# Autodesk Inventor assembly: AM14U3 Long Frame Half
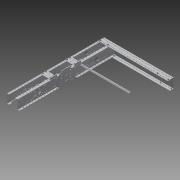
[picture p0: Inventor's stored thumbnail of the model, 180x180]
Saved by Autodesk Inventor 2018 (Build 220112000, 112)
## iProperties
Created: 2015-12-05
Part Number: AM14U3 Long Frame Half
Document SubType Name: Assembly
Designer: PhillipD
Author: PhillipD
Revision Number: ANY
## Documents named in this file (9)
- D:\FIRST 2018\FIRST 2018 Inventor\FIRST 2017 Drive Base\Parts\AM14U3 Long Frame Half.iam
- D:\FIRST 2018\FIRST 2018 Inventor\FIRST 2017 Drive Base\Parts\Churro 3375.ipt
- D:\FIRST 2018\FIRST 2018 Inventor\FIRST 2017 Drive Base\Parts\FHTS 0.25-20-0.75_FHTS 0.25-20-G-0.75-C.ipt
- D:\FIRST 2018\FIRST 2018 Inventor\FIRST 2017 Drive Base\Parts\AM14U3 End Sheet Long.ipt
- D:\FIRST 2018\FIRST 2018 Inventor\FIRST 2017 Drive Base\Parts\AM14U3 Inside Sheet Rev2.ipt
- D:\FIRST 2018\FIRST 2018 Inventor\FIRST 2017 Drive Base\Parts\AM14U3 Outside Sheet Rev1_DefaultSM-FLAT-PATTERN.ipt
- D:\FIRST 2018\FIRST 2018 Inventor\FIRST 2017 Drive Base\Parts\am-2954 AM14U2 2x3 Hole Bracket.ipt
- D:\FIRST 2018\FIRST 2018 Inventor\FIRST 2017 Drive Base\Parts\Churro 16250.ipt
- D:\FIRST 2018\FIRST 2018 Inventor\FIRST 2017 Drive Base\Parts\Nut_Screw.iam
## Components (40 placed, 21 different names)
1. Churro 3375_120
2. Churro 3375_121
3. Churro 3375_122
4. Churro 3375_123
5. FHTS 0.25-20-0.75_FHTS 0.25-20-G-0.75-C_125
6. FHTS 0.25-20-0.75_FHTS 0.25-20-G-0.75-C_126
7. FHTS 0.25-20-0.75_FHTS 0.25-20-G-0.75-C_127
8. FHTS 0.25-20-0.75_FHTS 0.25-20-G-0.75-C_128
9. FHTS 0.25-20-0.75_FHTS 0.25-20-G-0.75-C_129
10. FHTS 0.25-20-0.75_FHTS 0.25-20-G-0.75-C_130
11. FHTS 0.25-20-0.75_FHTS 0.25-20-G-0.75-C_131
12. FHTS 0.25-20-0.75_FHTS 0.25-20-G-0.75-C_132
13. FHTS 0.25-20-0.75_FHTS 0.25-20-G-0.75-C_133
14. FHTS 0.25-20-0.75_FHTS 0.25-20-G-0.75-C_134 — Mate:1, Mate:2
15. AM14U3 End Sheet Long_135 — Insert:14, Insert:15, Insert:16, Insert:17, Insert:18, Insert:19, Insert:20, Insert:21
16. AM14U3 Inside Sheet Rev2_136 — Insert:1, Insert:3, Insert:4, Insert:8, Insert:9, Insert:12, Insert:13
17. AM14U3 Outside Sheet Rev1_DefaultSM-FLAT-PATTERN_137 — Insert:2, Insert:5, Insert:6, Insert:7, Insert:10, Insert:11
18. am-2954 AM14U2 2x3 Hole Bracket_138
19. am-2954 AM14U2 2x3 Hole Bracket_139
20. Churro 16250:1 — Insert:1, Mate:1, Mate:2
21. Nut_Screw:2 [sub-assembly] — Insert:2
22. Nut_Screw:3 [sub-assembly] — Insert:3
23. Nut_Screw:4 [sub-assembly] — Insert:4
24. Nut_Screw:5 [sub-assembly] — Insert:5
25. Nut_Screw:6 [sub-assembly] — Insert:6
26. Nut_Screw:7 [sub-assembly] — Insert:7
27. Nut_Screw:8 [sub-assembly] — Insert:8
28. Nut_Screw:9 [sub-assembly] — Insert:9
29. Nut_Screw:10 [sub-assembly] — Insert:10
30. Nut_Screw:11 [sub-assembly] — Insert:11
31. Nut_Screw:12 [sub-assembly] — Insert:12
32. Nut_Screw:13 [sub-assembly] — Insert:13
33. Nut_Screw:14 [sub-assembly] — Insert:14
34. Nut_Screw:15 [sub-assembly] — Insert:15
35. Nut_Screw:16 [sub-assembly] — Insert:16
36. Nut_Screw:17 [sub-assembly] — Insert:17
37. Nut_Screw:18 [sub-assembly] — Insert:18
38. Nut_Screw:19 [sub-assembly] — Insert:19
39. Nut_Screw:20 [sub-assembly] — Insert:20
40. Nut_Screw:21 [sub-assembly] — Insert:21
## Relationships (23: Insert 21, Mate 2)
- Insert:1: AM14U3 Inside Sheet Rev2_136 ↔ Churro 16250:1
- Mate:1: FHTS 0.25-20-0.75_FHTS 0.25-20-G-0.75-C_134 ↔ Churro 16250:1
- Mate:2 (3.175 mm): FHTS 0.25-20-0.75_FHTS 0.25-20-G-0.75-C_134 ↔ Churro 16250:1
- Insert:2: AM14U3 Outside Sheet Rev1_DefaultSM-FLAT-PATTERN_137 ↔ Nut_Screw:2
- Insert:3: AM14U3 Inside Sheet Rev2_136 ↔ Nut_Screw:3
- Insert:4: AM14U3 Inside Sheet Rev2_136 ↔ Nut_Screw:4
- Insert:5: AM14U3 Outside Sheet Rev1_DefaultSM-FLAT-PATTERN_137 ↔ Nut_Screw:5
- Insert:6: AM14U3 Outside Sheet Rev1_DefaultSM-FLAT-PATTERN_137 ↔ Nut_Screw:6
- Insert:7: AM14U3 Outside Sheet Rev1_DefaultSM-FLAT-PATTERN_137 ↔ Nut_Screw:7
- Insert:8: AM14U3 Inside Sheet Rev2_136 ↔ Nut_Screw:8
- Insert:9: AM14U3 Inside Sheet Rev2_136 ↔ Nut_Screw:9
- Insert:10: AM14U3 Outside Sheet Rev1_DefaultSM-FLAT-PATTERN_137 ↔ Nut_Screw:10
- Insert:11: AM14U3 Outside Sheet Rev1_DefaultSM-FLAT-PATTERN_137 ↔ Nut_Screw:11
- Insert:12: AM14U3 Inside Sheet Rev2_136 ↔ Nut_Screw:12
- Insert:13: AM14U3 Inside Sheet Rev2_136 ↔ Nut_Screw:13
- Insert:14: AM14U3 End Sheet Long_135 ↔ Nut_Screw:14
- Insert:15: AM14U3 End Sheet Long_135 ↔ Nut_Screw:15
- Insert:16: AM14U3 End Sheet Long_135 ↔ Nut_Screw:16
- Insert:17: AM14U3 End Sheet Long_135 ↔ Nut_Screw:17
- Insert:18: AM14U3 End Sheet Long_135 ↔ Nut_Screw:18
- Insert:19: AM14U3 End Sheet Long_135 ↔ Nut_Screw:19
- Insert:20: AM14U3 End Sheet Long_135 ↔ Nut_Screw:20
- Insert:21: AM14U3 End Sheet Long_135 ↔ Nut_Screw:21
